# Autodesk Inventor assembly: A600 Keyboard
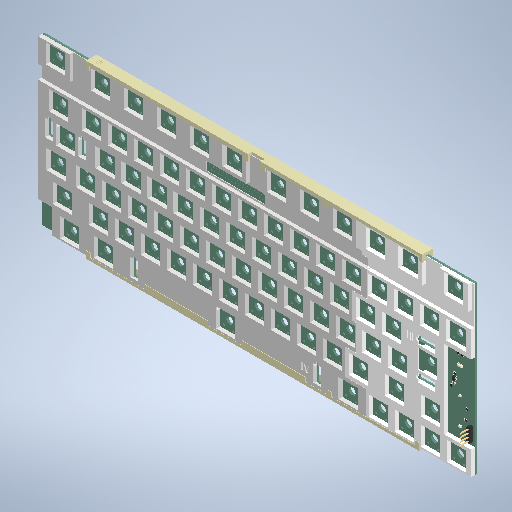
[picture p0: Inventor's stored thumbnail of the model, 512x512]
Saved by Autodesk Inventor 2025.1 (Build 291241000, 241)
## iProperties
Created: 2024-08-15
Part Number: A600 Keyboard
Document SubType Name: Assembly
Designer: adam
Author: adam
## Documents named in this file (6)
- C:\Users\adam\Projects\A600KBv2\3dprint\Keyboard Plates\A600 Keyboard.iam
- C:\Users\adam\Projects\A600KBv2\3dprint\Keyboard Plates\A600KBv3\A600KBv3.ipt
- C:\Users\adam\Projects\A600KBv2\3dprint\Keyboard Plates\Left Plate.ipt
- C:\Users\adam\Projects\A600KBv2\3dprint\Keyboard Plates\Right Plate.ipt
- C:\Users\adam\Projects\A600KBv2\3dprint\Keyboard Plates\Case Rail.ipt
- C:\Users\adam\Projects\A600KBv2\3dprint\Keyboard Plates\Top Case Rail.ipt
## Components (5 placed, 5 different names)
1. A600KBv3:1 — Flush:1, Flush:2, Mate:1, Mate:3
2. Left Plate:1 — Flush:1, Flush:3, Mate:2, Flush:4, Mate:4
3. Right Plate:1 — Flush:2
4. Case Rail:1 — Mate:3, Flush:4, Mate:4
5. Top Case Rail:1 — Flush:3, Mate:1, Mate:2
## Relationships (8: Flush 4, Mate 4)
- Flush:1: A600KBv3:1 ↔ Left Plate:1
- Flush:2: A600KBv3:1 ↔ Right Plate:1
- Flush:3: Left Plate:1 ↔ Top Case Rail:1
- Mate:1: A600KBv3:1 ↔ Top Case Rail:1
- Mate:2: Left Plate:1 ↔ Top Case Rail:1
- Mate:3: A600KBv3:1 ↔ Case Rail:1
- Flush:4: Left Plate:1 ↔ Case Rail:1
- Mate:4: Left Plate:1 ↔ Case Rail:1
